# Autodesk Inventor assembly: Сборка3
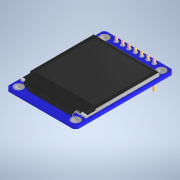
[picture p0: Inventor's stored thumbnail of the model, 180x180]
Saved by Autodesk Inventor 2020 (Build 240168000, 168)
## iProperties
Created: 2021-09-23
Part Number: Сборка3
Document SubType Name: Assembly
Designer: Andrei
Author: Andrei
## Documents named in this file (3)
- C:\Users\Andre\Desktop\Новая папка\Сборка3.iam
- C:\Users\Andre\Desktop\Новая папка\1.3 TFT IPS - Flush Reverse Mount(1).ipt
- C:\Users\Andre\Desktop\Новая папка\Деталь12.ipt
## Components (2 placed, 2 different names)
1. Деталь12:1 — Совмещение:1
2. 1.3 TFT IPS - Flush Reverse Mount(1):1 — Совмещение:1
## Relationships (1: Mate 1)
- Совмещение:1 [Mate]: Деталь12:1 ↔ 1.3 TFT IPS - Flush Reverse Mount(1):1
